# Autodesk Inventor assembly: chassisv2
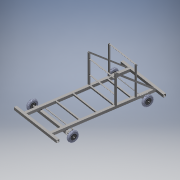
[picture p0: Inventor's stored thumbnail of the model, 180x180]
Saved by Autodesk Inventor 2018 (Build 220112000, 112)
## iProperties
Created: 2018-08-06
Part Number: chassisv2
Document SubType Name: Assembly
Designer: Cole Tucker
Mass: 65054.1 g
Surface Area: 48005.5 cm^2
Volume: 9918.17 cm^3
Density: 6.55908 g/cm^3
Author: Cole Tucker
## Documents named in this file (12)
- C:\Users\Cole Tucker\Documents\Github\2018-Personal-Robot\CAD\chassis\Inventor\chassisv2.iam
- C:\Users\Cole Tucker\Documents\Github\2018-Personal-Robot\CAD\chassis\Inventor\framev2.iam
- C:\Users\Cole Tucker\Documents\Github\2018-Personal-Robot\CAD\chassis\Inventor\chassisv2\Design Accelerator\Shaft2.iam
- C:\Users\Cole Tucker\Documents\Github\2018-Personal-Robot\CAD\chassis\Inventor\chassisv2\Design Accelerator\Bearing1.iam
- C:\Users\Cole Tucker\Documents\Github\2018-Personal-Robot\CAD\chassis\Inventor\steeringarm.iam
- C:\Users\Cole Tucker\Documents\Inventor\Content Center Files\R2018\en-US\ANSI B18.2.1(3)\ANSI B18.2.1 - 3_8-16 UNC - 1.25(3).ipt
- C:\Users\Cole Tucker\Documents\Inventor\Content Center Files\R2018\en-US\ANSI B18.2.2(09)\ANSI B18.2.2 - 3_8 - 24(2).ipt
- C:\Users\Cole Tucker\Documents\Github\2018-Personal-Robot\CAD\chassis\Inventor\PneumaticWheel_am-0970.iam
- C:\Users\Cole Tucker\Documents\Github\2018-Personal-Robot\CAD\chassis\Inventor\am-0077a-500 Key Hub r2.ipt
- C:\Users\Cole Tucker\Documents\Inventor\Content Center Files\R2018\en-US\ANSI B18.2.1(3)\ANSI B18.2.1 - 3_8-16 UNC - 2.75(3).ipt
- C:\Users\Cole Tucker\Documents\Github\2018-Personal-Robot\CAD\chassis\Inventor\steeringlinkage.ipt
- steeringarm.ipt
## Components (25 placed, 10 different names)
1. framev2:1 [sub-assembly] — Mate:1, Flush:1, Mate:3, Flush:2, Mate:4, Mate:7, Mate:8, Mate:96, Mate:102, Mate:103, Mate:105, Mate:107, Mate:109, Mate:111
2. Shaft:1 [sub-assembly] — Mate:1, Flush:1, Mate:2, Mate:78, Flush:10, Mate:82, Flush:11
3. Bearing:1 [sub-assembly] — Mate:2, Mate:3
4. Bearing:2 [sub-assembly] — Flush:2, Mate:4
5. steeringarm:1 [sub-assembly] — Mate:7, Mate:8, Mate:74, Flush:9, Mate:91, Mate:93, Mate:104
6. steeringarm:2 [sub-assembly] — Mate:71, Flush:6, Mate:96, Mate:97, Mate:99, Mate:101, Mate:106, Mate:113
7. Hex Cap Screw - Inch 3/8-16 UNC - 1.25:2 — Mate:62, Mate:97, Mate:101, Mate:112
8. Hex Cap Screw - Inch 3/8-16 UNC - 1.25:1 — Mate:65, Mate:91, Mate:104, Mate:114
9. Hex Nut - Inch 3/8 - 24:1 — Mate:65, Mate:93
10. Hex Nut - Inch 3/8 - 24:2 — Mate:62, Mate:99
11. Bearing:3 [sub-assembly] — Mate:69, Flush:4, Flush:6
12. Bearing:4 [sub-assembly] — Mate:70, Flush:5, Mate:71
13. Bearing:5 [sub-assembly] — Flush:7, Mate:72
14. Bearing:6 [sub-assembly] — Mate:73, Flush:8, Mate:74, Flush:9
15. PneumaticWheel_am-0970:1 [sub-assembly] — Mate:79, Mate:80, Mate:81, Flush:11
16. PneumaticWheel_am-0970:2 [sub-assembly] — Mate:75, Mate:76, Mate:77, Mate:78, Flush:10
17. PneumaticWheel_am-0970:3 [sub-assembly] — Flush:7, Mate:72, Mate:73, Flush:8
18. PneumaticWheel_am-0970:4 [sub-assembly] — Mate:69, Flush:4, Mate:70, Flush:5
19. am-0077a-500 Key Hub r2:1 — Mate:75, Mate:76, Mate:77
20. am-0077a-500 Key Hub r2:2 — Mate:79, Mate:80, Mate:81, Mate:82
21. Hex Cap Screw - Inch 3/8-16 UNC - 2.75:1 — Mate:102, Mate:103, Mate:110
22. Hex Cap Screw - Inch 3/8-16 UNC - 2.75:2 — Mate:105, Mate:106, Mate:107, Mate:108
23. Hex Nut - Inch 3/8 - 24:3 — Mate:108, Mate:109
24. Hex Nut - Inch 3/8 - 24:4 — Mate:110, Mate:111
25. steeringlinkage:1 — Mate:112, Mate:113, Mate:114
## Relationships (51: Mate 41, Flush 10)
- Mate:1: framev2:1 ↔ Shaft:1
- Flush:1 (-116.84 mm): framev2:1 ↔ Shaft:1
- Mate:2: Shaft:1 ↔ Bearing:1
- Mate:3: framev2:1 ↔ Bearing:1
- Flush:2: framev2:1 ↔ Bearing:2
- Mate:4: framev2:1 ↔ Bearing:2
- Mate:7: framev2:1 ↔ steeringarm:1
- Mate:8 (12.7 mm): framev2:1 ↔ steeringarm:1
- Mate:62: Hex Cap Screw - Inch 3/8-16 UNC - 1.25:2 ↔ Hex Nut - Inch 3/8 - 24:2
- Mate:65: Hex Cap Screw - Inch 3/8-16 UNC - 1.25:1 ↔ Hex Nut - Inch 3/8 - 24:1
- Mate:69: Bearing:3 ↔ PneumaticWheel_am-0970:4
- Flush:4: Bearing:3 ↔ PneumaticWheel_am-0970:4
- Mate:70: Bearing:4 ↔ PneumaticWheel_am-0970:4
- Flush:5: Bearing:4 ↔ PneumaticWheel_am-0970:4
- Mate:71: steeringarm:2 ↔ Bearing:4
- Flush:6 (-25.4 mm): steeringarm:2 ↔ Bearing:3
- Flush:7: Bearing:5 ↔ PneumaticWheel_am-0970:3
- Mate:72: Bearing:5 ↔ PneumaticWheel_am-0970:3
- Mate:73: Bearing:6 ↔ PneumaticWheel_am-0970:3
- Flush:8: Bearing:6 ↔ PneumaticWheel_am-0970:3
- Mate:74: steeringarm:1 ↔ Bearing:6
- Flush:9 (25.4 mm): steeringarm:1 ↔ Bearing:6
- Mate:75: PneumaticWheel_am-0970:2 ↔ am-0077a-500 Key Hub r2:1
- Mate:76: PneumaticWheel_am-0970:2 ↔ am-0077a-500 Key Hub r2:1
- Mate:77: PneumaticWheel_am-0970:2 ↔ am-0077a-500 Key Hub r2:1
- Mate:78: Shaft:1 ↔ PneumaticWheel_am-0970:2
- Flush:10 (-25.4 mm): Shaft:1 ↔ PneumaticWheel_am-0970:2
- Mate:79: PneumaticWheel_am-0970:1 ↔ am-0077a-500 Key Hub r2:2
- Mate:80: PneumaticWheel_am-0970:1 ↔ am-0077a-500 Key Hub r2:2
- Mate:81: PneumaticWheel_am-0970:1 ↔ am-0077a-500 Key Hub r2:2
- Mate:82: Shaft:1 ↔ am-0077a-500 Key Hub r2:2
- Flush:11 (25.4 mm): Shaft:1 ↔ PneumaticWheel_am-0970:1
- Mate:91: steeringarm:1 ↔ Hex Cap Screw - Inch 3/8-16 UNC - 1.25:1
- Mate:93: steeringarm:1 ↔ Hex Nut - Inch 3/8 - 24:1
- Mate:96 (12.7 mm): framev2:1 ↔ steeringarm:2
- Mate:97: steeringarm:2 ↔ Hex Cap Screw - Inch 3/8-16 UNC - 1.25:2
- Mate:99: steeringarm:2 ↔ Hex Nut - Inch 3/8 - 24:2
- Mate:101 (6.35 mm): steeringarm:2 ↔ Hex Cap Screw - Inch 3/8-16 UNC - 1.25:2
- Mate:102: framev2:1 ↔ Hex Cap Screw - Inch 3/8-16 UNC - 2.75:1
- Mate:103: framev2:1 ↔ Hex Cap Screw - Inch 3/8-16 UNC - 2.75:1
- Mate:104 (6.35 mm): steeringarm:1 ↔ Hex Cap Screw - Inch 3/8-16 UNC - 1.25:1
- Mate:105: framev2:1 ↔ Hex Cap Screw - Inch 3/8-16 UNC - 2.75:2
- Mate:106: steeringarm:2 ↔ Hex Cap Screw - Inch 3/8-16 UNC - 2.75:2
- Mate:107: framev2:1 ↔ Hex Cap Screw - Inch 3/8-16 UNC - 2.75:2
- Mate:108: Hex Cap Screw - Inch 3/8-16 UNC - 2.75:2 ↔ Hex Nut - Inch 3/8 - 24:3
- Mate:109: framev2:1 ↔ Hex Nut - Inch 3/8 - 24:3
- Mate:110: Hex Cap Screw - Inch 3/8-16 UNC - 2.75:1 ↔ Hex Nut - Inch 3/8 - 24:4
- Mate:111: framev2:1 ↔ Hex Nut - Inch 3/8 - 24:4
- Mate:112: Hex Cap Screw - Inch 3/8-16 UNC - 1.25:2 ↔ steeringlinkage:1
- Mate:113: steeringarm:2 ↔ steeringlinkage:1
- Mate:114: Hex Cap Screw - Inch 3/8-16 UNC - 1.25:1 ↔ steeringlinkage:1
